# Autodesk Inventor assembly: CollectorArmWWheelAssembly
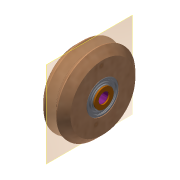
[picture p0: Inventor's stored thumbnail of the model, 180x180]
Saved by Autodesk Inventor 2018 (Build 220112000, 112)
## iProperties
Created: 2018-11-25
Part Number: CollectorArmWWheelAssembly
Document SubType Name: Assembly
Designer: ball
Author: ball
## Documents named in this file (4)
- C:\FTC\FTC8863CAD\2018Robot\CollectorArmWWheelAssembly.iam
- C:\FTC\FTC8863CAD\GoBilda\3600 Parts\3600-0006-2910 Assembly.ipt
- C:\FTC\FTC8863CAD\GoBilda\2807 Parts\2807-0407-0500.ipt
- C:\FTC\FTC8863CAD\GoBilda\1502 Parts\1502-0006-0100.ipt
## Components (3 placed, 3 different names)
1. 3600-0006-2910 Assembly:1 — Mate:1, Mate:2, Flush:1, Mate:3
2. 2807-0407-0500:1 — Mate:1, Mate:2
3. 1502-0006-0100:2 — Flush:1, Mate:3
## Relationships (4: Mate 3, Flush 1)
- Mate:1: 3600-0006-2910 Assembly:1 ↔ 2807-0407-0500:1
- Mate:2: 3600-0006-2910 Assembly:1 ↔ 2807-0407-0500:1
- Flush:1: 3600-0006-2910 Assembly:1 ↔ 1502-0006-0100:2
- Mate:3: 3600-0006-2910 Assembly:1 ↔ 1502-0006-0100:2
